# Autodesk Inventor assembly: 2016-02-02-RhinoRobotV08
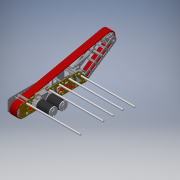
[picture p0: Inventor's stored thumbnail of the model, 180x180]
Saved by Autodesk Inventor 2016 SP1 (Build 200210100, 210)
## iProperties
Created: 2016-01-23
Part Number: 2016-02-02-RhinoRobotV08
Document SubType Name: Assembly
Designer: steele
Mass: 23360.3 g
Surface Area: 43274.3 cm^2
Volume: 23034.6 cm^3
Density: 1.01414 g/cm^3
Author: steele
## Documents named in this file (8)
- C:\snobotics\CAD-Development\robSteele\SnoBotics2016\2016-02-04-RhinoRobotNarrowVersion\2016-02-02-RhinoRobotV08.iam
- C:\snobotics\CAD-Development\robSteele\SnoBotics2016\RhinoTrackDriveModule\am-3322+RhinoTrackDriveModule.iam
- C:\snobotics\CAD-Development\robSteele\SnoBotics2016\RhinoBottomFloorOptions\RhinoBottomFloorPlate01.ipt
- C:\snobotics\CAD-Development\robSteele\SnoBotics2016\RhinoTrackDriveModule\am-3322+RhinoTrackDriveModule_MIR9.iam
- C:\snobotics\CAD-Development\robSteele\SnoBotics2016\RhinoBottomFloorOptions\RhinoBottomFloorPlate05.ipt
- C:\snobotics\CAD-Development\robSteele\SnoBotics2016\2016-01-31-Lift\2016-01-31-LiftTiltAssembly.iam
- C:\snobotics\CAD-Development\robSteele\SnoBotics2016\AM Parts\Churo_16_5_inches.ipt
- C:\snobotics\CAD-Development\robSteele\SnoBotics2016\2016-02-04-RhinoRobotNarrowVersion\2016-02-02-RhinoRobotV08\Design Accelerator\Bolted Connection2.iam
## Components (11 placed, 7 different names)
1. RhinoBottomFloorPlate01:1 — Mate:1, Flush:2, Flush:11, Flush:14, Mate:18, Flush:15
2. am-3322+RhinoTrackDriveModule:1 [sub-assembly] — Mate:1, Flush:2, Flush:11, Flush:12, Flush:13, Mate:17, Insert:1, Mate:19, Insert:2, Insert:3, Insert:4, Insert:5
3. am-3322+RhinoTrackDriveModule_MIR9:1 [sub-assembly]
4. RhinoBottomFloorPlate05:1 — Flush:12, Flush:13, Mate:17
5. 2016-01-31-LiftTiltAssembly:1 [sub-assembly] — Flush:14, Mate:18, Flush:15
6. Churo_16_5_inches:1 — Insert:1, Mate:20
7. Bolted Connection:1 [sub-assembly] — Mate:19, Mate:20
8. Churo_16_5_inches:2 — Insert:2
9. Churo_16_5_inches:3 — Insert:3
10. Churo_16_5_inches:4 — Insert:4
11. Churo_16_5_inches:5 — Insert:5
## Relationships (16: Flush 6, Mate 5, Insert 5)
- Mate:1: RhinoBottomFloorPlate01:1 ↔ am-3322+RhinoTrackDriveModule:1
- Flush:2: RhinoBottomFloorPlate01:1 ↔ am-3322+RhinoTrackDriveModule:1
- Flush:11: RhinoBottomFloorPlate01:1 ↔ am-3322+RhinoTrackDriveModule:1
- Flush:12: am-3322+RhinoTrackDriveModule:1 ↔ RhinoBottomFloorPlate05:1
- Flush:13: am-3322+RhinoTrackDriveModule:1 ↔ RhinoBottomFloorPlate05:1
- Mate:17: am-3322+RhinoTrackDriveModule:1 ↔ RhinoBottomFloorPlate05:1
- Flush:14: RhinoBottomFloorPlate01:1 ↔ 2016-01-31-LiftTiltAssembly:1
- Mate:18: RhinoBottomFloorPlate01:1 ↔ 2016-01-31-LiftTiltAssembly:1
- Flush:15: RhinoBottomFloorPlate01:1 ↔ 2016-01-31-LiftTiltAssembly:1
- Insert:1: am-3322+RhinoTrackDriveModule:1 ↔ Churo_16_5_inches:1
- Mate:19: am-3322+RhinoTrackDriveModule:1 ↔ Bolted Connection:1
- Mate:20: Churo_16_5_inches:1 ↔ Bolted Connection:1
- Insert:2: am-3322+RhinoTrackDriveModule:1 ↔ Churo_16_5_inches:2
- Insert:3: am-3322+RhinoTrackDriveModule:1 ↔ Churo_16_5_inches:3
- Insert:4: am-3322+RhinoTrackDriveModule:1 ↔ Churo_16_5_inches:4
- Insert:5: am-3322+RhinoTrackDriveModule:1 ↔ Churo_16_5_inches:5
## Named parameters: robotWidth = 660.4 mm, halfRobotWidth = 330.2 mm, maxPerimeter = 3048 mm, maxLength = 863.6 mm, widthOfTrack = 95.25 mm, boardWidth = 469.9 mm
